# Autodesk Inventor assembly: 2110_Position Assm_V1
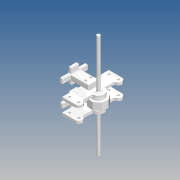
[picture p0: Inventor's stored thumbnail of the model, 180x180]
Saved by Autodesk Inventor 2020 (Build 240168000, 168)
## iProperties
Created: 2019-11-20
Part Number: 2110_Position Assm_V1
Document SubType Name: Assembly
Designer: RFLab
Author: RFLab
## Documents named in this file (5)
- C:\Users\RFLab\Dropbox\MPI Group Folder\MPS\Inventor_Parts\Parts Numbered - OSMPI\2xxx_Sample Holder and Rx\21xx_Rx Coil Assembly\2110_Position Assm_V1.iam
- C:\Users\RFLab\Dropbox\MPI Group Folder\MPS\Inventor_Parts\MPS System Assembly\V2\2019_11_08_threaded_rod.ipt
- C:\Users\RFLab\Dropbox\MPI Group Folder\MPS\Inventor_Parts\MPS System Assembly\V2\2019_11_20_fix_position_nut.ipt
- C:\Users\RFLab\Dropbox\MPI Group Folder\MPS\Inventor_Parts\Parts Numbered - OSMPI\2xxx_Sample Holder and Rx\21xx_Rx Coil Assembly\2112_Adjustment Nut_V1.ipt
- C:\Users\RFLab\Dropbox\MPI Group Folder\MPS\Inventor_Parts\Parts Numbered - OSMPI\2xxx_Sample Holder and Rx\21xx_Rx Coil Assembly\2113_Nut Stop Plate_V1.ipt
## Components (6 placed, 4 different names)
1. 2112_Adjustment Nut_V1:1 — Mate:1, Mate:5, Mate:6
2. 2019_11_08_threaded_rod:1 — Mate:1, Mate:2, Mate:3
3. 2113_Nut Stop Plate_V1:1 — Mate:3, Mate:5, Mate:7, Mate:8, Mate:9, Mate:13, Mate:16
4. 2113_Nut Stop Plate_V1:2 — Mate:2, Mate:6, Mate:10, Mate:11, Mate:12, Mate:13, Flush:1
5. 2019_11_20_fix_position_nut:1 — Mate:7, Mate:8, Mate:9, Mate:14, Mate:15
6. 2019_11_20_fix_position_nut:2 — Mate:10, Mate:11, Mate:12
## Relationships (16: Mate 15, Flush 1)
- Mate:1: 2112_Adjustment Nut_V1:1 ↔ 2019_11_08_threaded_rod:1
- Mate:2: 2019_11_08_threaded_rod:1 ↔ 2113_Nut Stop Plate_V1:2
- Mate:3: 2019_11_08_threaded_rod:1 ↔ 2113_Nut Stop Plate_V1:1
- Mate:5 (1 mm): 2112_Adjustment Nut_V1:1 ↔ 2113_Nut Stop Plate_V1:1
- Mate:6 (1 mm): 2112_Adjustment Nut_V1:1 ↔ 2113_Nut Stop Plate_V1:2
- Mate:7: 2113_Nut Stop Plate_V1:1 ↔ 2019_11_20_fix_position_nut:1
- Mate:8: 2113_Nut Stop Plate_V1:1 ↔ 2019_11_20_fix_position_nut:1
- Mate:9: 2113_Nut Stop Plate_V1:1 ↔ 2019_11_20_fix_position_nut:1
- Mate:10: 2113_Nut Stop Plate_V1:2 ↔ 2019_11_20_fix_position_nut:2
- Mate:11: 2113_Nut Stop Plate_V1:2 ↔ 2019_11_20_fix_position_nut:2
- Mate:12: 2113_Nut Stop Plate_V1:2 ↔ 2019_11_20_fix_position_nut:2
- Mate:13: 2113_Nut Stop Plate_V1:1 ↔ 2113_Nut Stop Plate_V1:2
- Mate:14: 2019_11_20_fix_position_nut:1
- Mate:15: 2019_11_20_fix_position_nut:1
- Mate:16: 2113_Nut Stop Plate_V1:1
- Flush:1: 2113_Nut Stop Plate_V1:2
